# Autodesk Inventor assembly: Motor_Section_MIR1
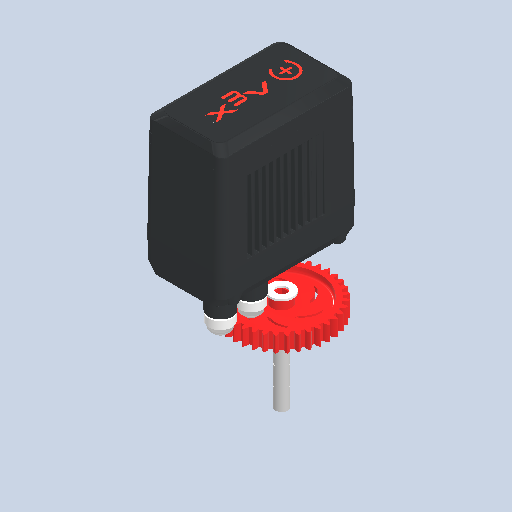
[picture p0: Inventor's stored thumbnail of the model, 512x512]
Saved by Autodesk Inventor 2025.2 (Build 292293000, 293)
## iProperties
Created: 2024-12-08
Part Number: Motor_Section_MIR1
Document SubType Name: Assembly
Designer: joshi
Author: Aditya Koduri
## Documents named in this file (10)
- C:\Users\joshi\Desktop\3388K CAD\Motor_Section_MIR1.iam
- C:\Users\joshi\Desktop\3388K CAD\VEX Main\Motion\Spacers\Washer Teflon\TWasher .375 OD x .03125.ipt
- C:\Users\joshi\Desktop\3388K CAD\VEX Main\Motion\Spacers\Washer Teflon.ipt
- C:\Users\joshi\Desktop\3388K CAD\VEX Main\Motion\Gears\LS 36T Gear_MIR1.ipt
- C:\Users\joshi\Desktop\3388K CAD\Thin_spacer_custom_MIR1.ipt
- C:\Users\joshi\Desktop\3388K CAD\VEX Main\Electronics\V5 Motor_MIR1.ipt
- C:\Users\joshi\Desktop\3388K CAD\VEX Main\Motion\Spacers\Spacer Nylon .313 OD\NSpacer .313 OD x .125.ipt
- C:\Users\joshi\Desktop\3388K CAD\VEX Main\Motion\Spacers\Spacer Nylon .313 OD.ipt
- C:\Users\joshi\Desktop\3388K CAD\VEX Main\Structure\Hardware\Screw Steel - Hex\SScrew Hex Smooth .500.ipt
- C:\Users\joshi\Desktop\3388K CAD\VEX Main\Structure\Hardware\Screw Steel - Hex.ipt
## Components (11 placed, 6 different names)
1. TWasher .375 OD x .03125:1 — Insert:1
2. LS 36T Gear_MIR1:1 — Insert:1, Insert:5
3. Thin_spacer_custom_MIR1:1 — Insert:2, Insert:3
4. Thin_spacer_custom_MIR1:2 — Insert:5, Insert:4
5. Thin_spacer_custom_MIR1:3 — Insert:2, Insert:4
6. Thin_spacer_custom_MIR1:4 — Insert:3
7. V5 Motor_MIR1:1 — Insert:6, Insert:7
8. NSpacer .313 OD x .125:1 — Insert:6
9. NSpacer .313 OD x .125:2 — Insert:7
10. SScrew Hex Smooth .500:1
11. SScrew Hex Smooth .500:2
## Relationships (7: Insert 7)
- Insert:1: TWasher .375 OD x .03125:1 ↔ LS 36T Gear_MIR1:1
- Insert:5: LS 36T Gear_MIR1:1 ↔ Thin_spacer_custom_MIR1:2
- Insert:2: Thin_spacer_custom_MIR1:1 ↔ Thin_spacer_custom_MIR1:3
- Insert:4: Thin_spacer_custom_MIR1:2 ↔ Thin_spacer_custom_MIR1:3
- Insert:3: Thin_spacer_custom_MIR1:1 ↔ Thin_spacer_custom_MIR1:4
- Insert:6: V5 Motor_MIR1:1 ↔ NSpacer .313 OD x .125:1
- Insert:7: V5 Motor_MIR1:1 ↔ NSpacer .313 OD x .125:2
